# Autodesk Inventor assembly: A_Airbert
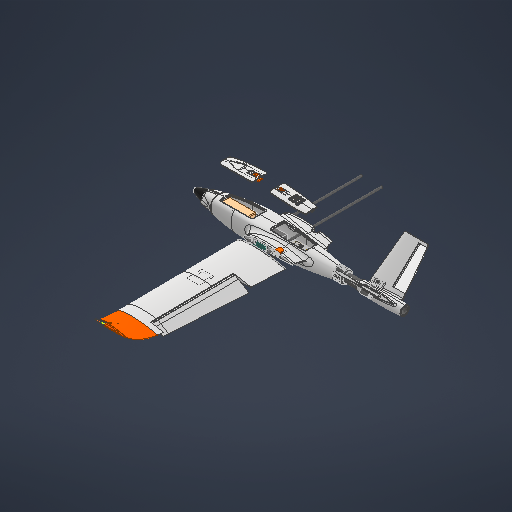
[picture p0: Inventor's stored thumbnail of the model, 512x512]
Saved by Autodesk Inventor 2026 (Build 300175000, 175)
## iProperties
Created: 2025-08-22
Part Number: A_Airbert
Document SubType Name: Assembly
Designer: FAL
Mass: 940.749 g
Surface Area: 6231.37 cm^2
Volume: 1491.38 cm^3
Author: FAL
## Documents named in this file (4)
- C:\Users\FAL\Projekte\Git\AIRBERT\CAD\A_Airbert.iam
- C:\Users\FAL\Projekte\Git\AIRBERT\CAD\Wing\A_Wing.iam
- C:\Users\FAL\Projekte\Git\AIRBERT\CAD\Fuselage\A_Fuselage.iam
- C:\Users\FAL\Projekte\Git\AIRBERT\CAD\Aft\A_Aft.iam
## Components (3 placed, 3 different names)
1. A_Wing:1 [sub-assembly] — Fluchtend:1, Fluchtend:2, Fluchtend:3
2. A_Fuselage:1 [sub-assembly] — Fluchtend:4, Fluchtend:5, Fluchtend:6
3. A_Aft:1 [sub-assembly] — Fluchtend:7, Fluchtend:8
## Relationships (8: Flush 8)
- Fluchtend:1 [Flush]: A_Wing:1
- Fluchtend:2 [Flush]: A_Wing:1
- Fluchtend:3 [Flush]: A_Wing:1
- Fluchtend:4 [Flush]: A_Fuselage:1
- Fluchtend:5 [Flush]: A_Fuselage:1
- Fluchtend:6 [Flush]: A_Fuselage:1
- Fluchtend:7 [Flush]: A_Aft:1
- Fluchtend:8 [Flush]: A_Aft:1
